# Autodesk Inventor assembly: bunny bot 2013 manipulator 3
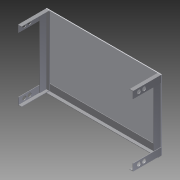
[picture p0: Inventor's stored thumbnail of the model, 180x180]
Saved by Autodesk Inventor 2012 (Build 160160000, 160)
## iProperties
Created: 2013-10-01
Part Number: bunny bot 2013 manipulator 3
Document SubType Name: Assembly
Designer: Bryce
Author: Bryce
## Documents named in this file (6)
- C:\Users\Bryce\Dropbox\Inventor Design Project Files\Independent Swerves\Inventor 2012\bunny bot 2013 manipulator 3.iam
- C:\Users\Bryce\Dropbox\Inventor Design Project Files\Independent Swerves\Inventor 2012\manipulator bearing back right.ipt
- C:\Users\Bryce\Dropbox\Inventor Design Project Files\Independent Swerves\Inventor 2012\manipulator bearing back left.ipt
- C:\Users\Bryce\Dropbox\Inventor Design Project Files\Independent Swerves\Inventor 2012\manipulator side L brace.ipt
- C:\Users\Bryce\Dropbox\Inventor Design Project Files\Independent Swerves\Inventor 2012\manipulator back L brace.ipt
- C:\Users\Bryce\Dropbox\Inventor Design Project Files\Independent Swerves\Inventor 2012\manipulator top.ipt
## Components (8 placed, 5 different names)
1. manipulator bearing back right:1 — Flush:1, Flush:2, Flush:3, Flush:5, Flush:7, Mate:1, Mate:2, Mate:5, Flush:8, Flush:10, Flush:11, Flush:12
2. manipulator bearing back right:2 — Flush:3, Flush:4, Flush:6
3. manipulator bearing back left:1 — Flush:5, Flush:6, Flush:7, Mate:1, Mate:4
4. manipulator bearing back left:2 — Flush:1, Flush:2, Flush:4, Mate:2, Mate:3, Mate:6, Flush:9, Mate:8
5. manipulator side L brace:1 — Mate:3, Mate:6, Flush:9, Mate:7
6. manipulator side L brace:2 — Mate:4, Mate:5, Flush:8, Mate:9
7. manipulator back L brace:1 — Mate:7, Mate:8, Flush:10
8. manipulator top:1 — Mate:9, Flush:11, Flush:12
## Relationships (21: Flush 12, Mate 9)
- Flush:1: manipulator bearing back right:1 ↔ manipulator bearing back left:2
- Flush:2: manipulator bearing back right:1 ↔ manipulator bearing back left:2
- Flush:3: manipulator bearing back right:1 ↔ manipulator bearing back right:2
- Flush:4: manipulator bearing back right:2 ↔ manipulator bearing back left:2
- Flush:5: manipulator bearing back right:1 ↔ manipulator bearing back left:1
- Flush:6: manipulator bearing back right:2 ↔ manipulator bearing back left:1
- Flush:7: manipulator bearing back right:1 ↔ manipulator bearing back left:1
- Mate:1 (-508 mm): manipulator bearing back right:1 ↔ manipulator bearing back left:1
- Mate:2 (-838.2 mm): manipulator bearing back right:1 ↔ manipulator bearing back left:2
- Mate:3: manipulator bearing back left:2 ↔ manipulator side L brace:1
- Mate:4: manipulator bearing back left:1 ↔ manipulator side L brace:2
- Mate:5: manipulator bearing back right:1 ↔ manipulator side L brace:2
- Mate:6: manipulator bearing back left:2 ↔ manipulator side L brace:1
- Flush:8: manipulator bearing back right:1 ↔ manipulator side L brace:2
- Flush:9: manipulator bearing back left:2 ↔ manipulator side L brace:1
- Mate:7: manipulator side L brace:1 ↔ manipulator back L brace:1
- Mate:8: manipulator bearing back left:2 ↔ manipulator back L brace:1
- Flush:10: manipulator bearing back right:1 ↔ manipulator back L brace:1
- Mate:9: manipulator side L brace:2 ↔ manipulator top:1
- Flush:11: manipulator bearing back right:1 ↔ manipulator top:1
- Flush:12: manipulator bearing back right:1 ↔ manipulator top:1
